# Autodesk Inventor assembly: Pier
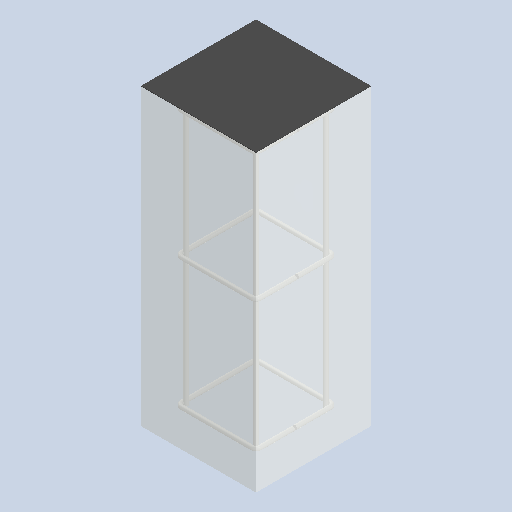
[picture p0: Inventor's stored thumbnail of the model, 512x512]
Saved by Autodesk Inventor 2025.1 (Build 291241020, 241B)
## iProperties
Created: 2024-09-15
Part Number: Pier
Document SubType Name: Assembly
Designer: Tom
Author: Tom
## Documents named in this file (4)
- C:\Users\Tom\Documents\Inventor\Mobility\Additional_Building\Pier.iam
- C:\Users\Tom\Documents\Inventor\Mobility\Additional_Building\Pier.ipt
- C:\Users\Tom\Documents\Inventor\Mobility\Additional_Building\Underlayment_For_Pier.ipt
- C:\Users\Tom\Documents\Inventor\Mobility\Additional_Building\Cage.iam
## Components (3 placed, 3 different names)
1. Pier:1 — Mate:1, Flush:1, Flush:2, Mate:2, Flush:3, Mate:3, Flush:4, Mate:4
2. Underlayment_For_Pier:1 — Mate:1, Flush:1, Flush:2
3. Cage:1 [sub-assembly] — Flush:4, Mate:4, Flush:5
## Relationships (9: Flush 5, Mate 4)
- Mate:1: Pier:1 ↔ Underlayment_For_Pier:1
- Flush:1: Pier:1 ↔ Underlayment_For_Pier:1
- Flush:2: Pier:1 ↔ Underlayment_For_Pier:1
- Mate:2: Pier:1
- Flush:3: Pier:1
- Mate:3: Pier:1
- Flush:4 (57.15 mm): Pier:1 ↔ Cage:1
- Mate:4 (-57.15 mm): Pier:1 ↔ Cage:1
- Flush:5: Cage:1
